# Autodesk Inventor assembly: Gobilda 1620 motor mount with motor
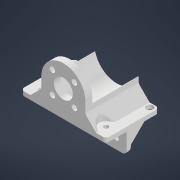
[picture p0: Inventor's stored thumbnail of the model, 180x180]
Saved by Autodesk Inventor 2022 (Build 260153000, 153)
## iProperties
Created: 2021-12-02
Part Number: Gobilda 1620 motor mount with motor
Document SubType Name: Assembly
Designer: izack
Author: izack
## Documents named in this file (3)
- F:\CAD Modeling\GithubCAD\ComputerAidedDesign\2021-22\FTC\#12456 Big Red\Drivetrain\Omni Wheel Drive\Gobilda 1620 motor mount with motor.iam
- F:\CAD Modeling\GithubCAD\ComputerAidedDesign\2021-22\FTC\#13822 Robovikes\Proof of Concept\13in^3 drivetrain parts\5202 Series Yellow Jacket Planetary Gear Motor.ipt
- F:\CAD Modeling\GithubCAD\ComputerAidedDesign\2021-22\FTC\#12456 Big Red\Drivetrain\Omni Wheel Drive\Gobilda 1620 motor mount.ipt
## Components (2 placed, 2 different names)
1. 5202 Series Yellow Jacket Planetary Gear Motor:1 — Flush:1
2. Gobilda 1620 motor mount:1 — Flush:1
## Relationships (1: Flush 1)
- Flush:1: 5202 Series Yellow Jacket Planetary Gear Motor:1 ↔ Gobilda 1620 motor mount:1
